# Autodesk Inventor assembly: ExteriorBumperCar
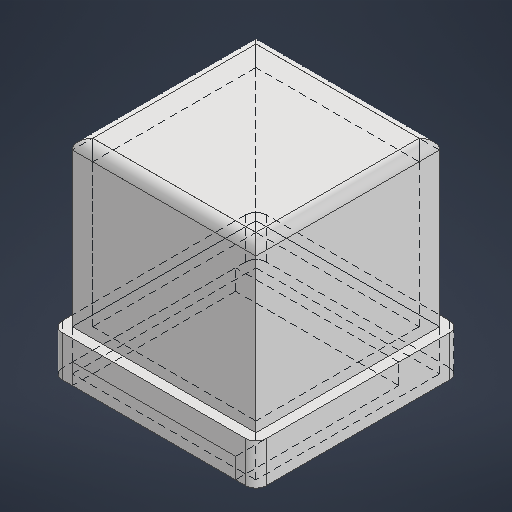
[picture p0: Inventor's stored thumbnail of the model, 512x512]
Saved by Autodesk Inventor 2026.1 (Build 301233000, 233)
## iProperties
Created: 2026-06-28
Part Number: ExteriorBumperCar
Document SubType Name: Assembly
Designer: Kasi Pusuluri
Author: Kasi Pusuluri
## Documents named in this file (3)
- C:\Users\Kasi Pusuluri\Documents\Outpost 2026\BumperCarV2\ExteriorBumperCar.iam
- C:\Users\Kasi Pusuluri\Documents\Outpost 2026\BumperCarV2\Top1.ipt
- C:\Users\Kasi Pusuluri\Documents\Outpost 2026\BumperCarV2\BumperBody.ipt
## Components (3 placed, 2 different names)
1. Top1:1 — Rigid:1
2. Top1:2 — Rigid:2
3. BumperBody:1 — Rigid:1, Rigid:2
## Relationships (2: WeldJoint 2)
- Rigid:1 [WeldJoint]: Top1:1 ↔ BumperBody:1
- Rigid:2 [WeldJoint]: Top1:2 ↔ BumperBody:1
